# Autodesk Inventor assembly: gate_not
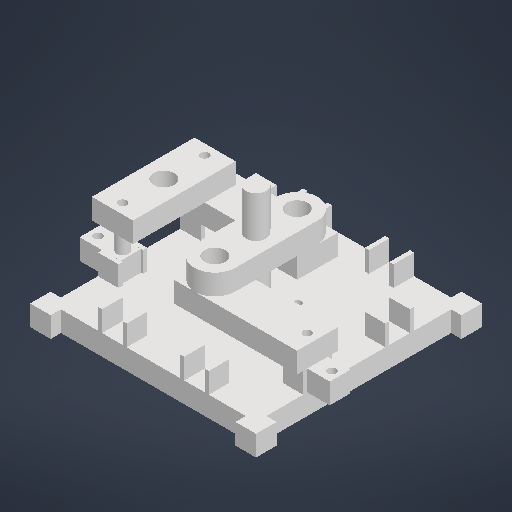
[picture p0: Inventor's stored thumbnail of the model, 512x512]
Saved by Autodesk Inventor 2025.4 (Build 294407000, 407)
## iProperties
Created: 2024-09-28
Part Number: gate_not
Document SubType Name: Assembly
Designer: sam
Author: sam
## Documents named in this file (8)
- G:\projects\secondary\computer_mechanical\gates\gate_not.iam
- G:\projects\secondary\computer_mechanical\gates\base.ipt
- G:\projects\secondary\computer_mechanical\gates\link.ipt
- G:\projects\secondary\computer_mechanical\gates\pin.ipt
- G:\projects\secondary\computer_mechanical\gates\block.ipt
- G:\projects\secondary\computer_mechanical\gates\link_small.ipt
- G:\projects\secondary\computer_mechanical\gates\bar.ipt
- G:\projects\secondary\computer_mechanical\gates\spacer_small.ipt
## Components (9 placed, 7 different names)
1. base:1 — Mate:16, Mate:17, Mate:29, Flush:1, Mate:34, Mate:35
2. link:2 — Mate:25, Mate:26, Mate:30, Mate:31, Mate:33
3. block:4 — Mate:16, Mate:17, Mate:23, Mate:24
4. link_small:1 — Mate:23, Mate:24, Mate:31, Mate:33
5. link_small:2 — Mate:25, Mate:26, Mate:32, Mate:38
6. pin:1 — Mate:29, Flush:1, Mate:30
7. block:5 — Mate:34, Mate:35, Mate:37, Mate:40, Flush:2
8. bar:1 — Mate:32, Mate:36, Mate:38, Mate:39, Flush:2
9. spacer_small:1 — Mate:36, Mate:37, Mate:39, Mate:40
## Relationships (20: Mate 18, Flush 2)
- Mate:16: base:1 ↔ block:4
- Mate:17: base:1 ↔ block:4
- Mate:23: block:4 ↔ link_small:1
- Mate:24: block:4 ↔ link_small:1
- Mate:25: link:2 ↔ link_small:2
- Mate:26: link:2 ↔ link_small:2
- Mate:29: base:1 ↔ pin:1
- Flush:1: base:1 ↔ pin:1
- Mate:30: link:2 ↔ pin:1
- Mate:31: link:2 ↔ link_small:1
- Mate:32: link_small:2 ↔ bar:1
- Mate:33: link:2 ↔ link_small:1
- Mate:34: base:1 ↔ block:5
- Mate:35: base:1 ↔ block:5
- Mate:36: bar:1 ↔ spacer_small:1
- Mate:37: block:5 ↔ spacer_small:1
- Mate:38: link_small:2 ↔ bar:1
- Mate:39: bar:1 ↔ spacer_small:1
- Mate:40: block:5 ↔ spacer_small:1
- Flush:2: block:5 ↔ bar:1
